# Autodesk Inventor assembly: solar_harvester_v2
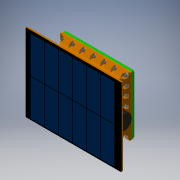
[picture p0: Inventor's stored thumbnail of the model, 180x180]
Saved by Autodesk Inventor 2018 (Build 220112000, 112)
## iProperties
Created: 2019-07-24
Part Number: solar_harvester_v2
Document SubType Name: Assembly
Designer: ZEUSLAP
Author: ZEUSLAP
## Documents named in this file (14)
- C:\data\solar-harvester\solar_harvester_136x110_CN3065_CGS.iam
- C:\data\solar-harvester\parts\sp16_waterproof_connector\sp16-2P_female_back_nut_type.iam
- C:\data\solar-harvester\parts\sp16_waterproof_connector\parts\nut.ipt
- C:\data\solar-harvester\parts\sp16_waterproof_connector\parts\rubber_washer.ipt
- C:\data\solar-harvester\enclosure\back\back_lid_CN3065_CGS.ipt
- C:\data\solar-harvester\parts\battery_holders\18650_battery_holder_CGS.ipt
- C:\data\solar-harvester\parts\18650_battery.ipt
- C:\data\solar-harvester\enclosure\back\charger_holder_CN3065.ipt
- C:\data\solar-harvester\enclosure\front\solar_panel_frame.ipt
- C:\data\solar-harvester\parts\panels\solar_panel_136x110mm.ipt
- C:\data\solar-harvester\parts\chargers\CN3065_solar_charger_board_Shrinkwrap.ipt
- C:\Users\ZEUSLAP\Documents\Inventor\Content Center Files\R2018\en-US\SFS EN ISO 7045 Z\EN ISO 7045 - M3 x 8 - 4.8 - Z(3).ipt
- C:\Users\ZEUSLAP\Documents\Inventor\Content Center Files\R2018\en-US\ISO 4035(2)\ISO 4035 - M3 - ISO.ipt
- C:\Users\ZEUSLAP\Documents\Inventor\Content Center Files\R2018\en-US\ISO 7049 - C-Z(2)\ISO 7049 - ST 2.9 x 6.5 - C - Z.ipt
## Components (59 placed, 13 different names)
1. solar_panel_136x110mm:1 — Mate:43, Mate:44, Angle:2, Mate:45
2. solar_panel_frame_136x110:1 — Mate:36, Mate:37, Mate:38, Angle:1, Mate:43, Mate:44, Angle:2, Mate:45, Mate:50, Mate:51, Mate:52, Mate:53, Angle:5, Mate:54, Mate:55, Mate:103, Mate:105, Mate:107, Mate:109, Mate:111, Mate:113, Mate:115, Mate:117, Mate:119, Mate:121, Mate:123, Mate:125, Mate:127, Mate:129, Mate:131, Mate:133, Mate:135, Mate:137, Mate:139, Mate:141, Mate:143, Mate:145, Mate:147
3. SP16-2P, female, back nut type:1 [sub-assembly] — Mate:31, Mate:32, Mate:34, Mate:37
4. nut:1 — Mate:32, Mate:38, Angle:1
5. rubber_washer:1 — Mate:31, Mate:34, Mate:36
6. back_lid_CN3065_CGS:1 — Mate:20, Mate:21, Mate:35, Mate:39, Angle:3, Angle:4, Mate:46, Mate:47, Mate:48, Mate:49, Mate:50, Mate:51, Mate:52, Mate:53, Mate:56, Mate:57, Mate:58, Mate:59, Mate:60, Mate:61, Mate:62, Mate:63, Mate:64, Mate:65, Mate:66, Mate:67, Mate:68, Mate:69, Mate:70, Mate:71, Mate:72, Mate:73, Mate:74, Mate:75, Mate:76, Mate:77, Mate:78, Mate:79, Mate:80, Mate:81, Mate:82, Mate:83, Mate:84, Mate:85, Mate:86, Mate:87, Mate:88, Mate:89, Mate:90, Mate:91, Mate:92, Mate:93, Mate:94, Mate:95, Mate:96, Mate:97, Mate:98, Mate:99, Mate:100, Mate:101, Mate:152
7. 18650_battery_holder_CGS:1 — Mate:22, Mate:23, Mate:35, Angle:3, Mate:46, Mate:153
8. 18650_battery:1 — Mate:22, Mate:23
9. CN3065_solar_charger_board:1 — Mate:39, Angle:4, Mate:48, Mate:49
10. charger_holder_CN3065:1 — Mate:20, Mate:21, Mate:47, Mate:148, Mate:149, Mate:150, Mate:151
11. SFS EN ISO 7045 Z M3 x 8 - 4.8 - Z:1 — Mate:56, Mate:57, Mate:108
12. SFS EN ISO 7045 Z M3 x 8 - 4.8 - Z:2 — Mate:58, Mate:59, Mate:118
13. SFS EN ISO 7045 Z M3 x 8 - 4.8 - Z:3 — Mate:60, Mate:61, Mate:122
14. SFS EN ISO 7045 Z M3 x 8 - 4.8 - Z:4 — Mate:62, Mate:63, Mate:138
15. SFS EN ISO 7045 Z M3 x 8 - 4.8 - Z:5 — Mate:64, Mate:65, Mate:142
16. SFS EN ISO 7045 Z M3 x 8 - 4.8 - Z:6 — Mate:66, Mate:67, Mate:136
17. SFS EN ISO 7045 Z M3 x 8 - 4.8 - Z:7 — Mate:68, Mate:69, Mate:132
18. SFS EN ISO 7045 Z M3 x 8 - 4.8 - Z:8 — Mate:70, Mate:71, Mate:128
19. SFS EN ISO 7045 Z M3 x 8 - 4.8 - Z:9 — Mate:72, Mate:73, Mate:124
20. SFS EN ISO 7045 Z M3 x 8 - 4.8 - Z:10 — Mate:74, Mate:75, Mate:112
21. SFS EN ISO 7045 Z M3 x 8 - 4.8 - Z:11 — Mate:76, Mate:77, Mate:104
22. SFS EN ISO 7045 Z M3 x 8 - 4.8 - Z:12 — Mate:78, Mate:79, Mate:102
23. SFS EN ISO 7045 Z M3 x 8 - 4.8 - Z:13 — Mate:80, Mate:81, Mate:106
24. SFS EN ISO 7045 Z M3 x 8 - 4.8 - Z:14 — Mate:82, Mate:83, Mate:110
25. SFS EN ISO 7045 Z M3 x 8 - 4.8 - Z:15 — Mate:84, Mate:85, Mate:114
26. SFS EN ISO 7045 Z M3 x 8 - 4.8 - Z:16 — Mate:86, Mate:87, Mate:126
27. SFS EN ISO 7045 Z M3 x 8 - 4.8 - Z:17 — Mate:88, Mate:89, Mate:130
28. SFS EN ISO 7045 Z M3 x 8 - 4.8 - Z:18 — Mate:90, Mate:91, Mate:134
29. SFS EN ISO 7045 Z M3 x 8 - 4.8 - Z:19 — Mate:92, Mate:93, Mate:144
30. SFS EN ISO 7045 Z M3 x 8 - 4.8 - Z:20 — Mate:94, Mate:95, Mate:140
31. SFS EN ISO 7045 Z M3 x 8 - 4.8 - Z:21 — Mate:96, Mate:97, Mate:146
32. SFS EN ISO 7045 Z M3 x 8 - 4.8 - Z:22 — Mate:98, Mate:99, Mate:120
33. SFS EN ISO 7045 Z M3 x 8 - 4.8 - Z:23 — Mate:100, Mate:101, Mate:116
34. ISO 4035 M3:1 — Mate:102, Mate:103
35. ISO 4035 M3:2 — Mate:104, Mate:105
36. ISO 4035 M3:3 — Mate:106, Mate:107
37. ISO 4035 M3:4 — Mate:108, Mate:109
38. ISO 4035 M3:5 — Mate:110, Mate:111
39. ISO 4035 M3:6 — Mate:112, Mate:113
40. ISO 4035 M3:7 — Mate:114, Mate:115
41. ISO 4035 M3:8 — Mate:116, Mate:117
42. ISO 4035 M3:9 — Mate:118, Mate:119
43. ISO 4035 M3:10 — Mate:120, Mate:121
44. ISO 4035 M3:11 — Mate:122, Mate:123
45. ISO 4035 M3:12 — Mate:124, Mate:125
46. ISO 4035 M3:13 — Mate:126, Mate:127
47. ISO 4035 M3:14 — Mate:128, Mate:129
48. ISO 4035 M3:15 — Mate:130, Mate:131
49. ISO 4035 M3:16 — Mate:132, Mate:133
50. ISO 4035 M3:17 — Mate:134, Mate:135
51. ISO 4035 M3:18 — Mate:136, Mate:137
52. ISO 4035 M3:19 — Mate:138, Mate:139
53. ISO 4035 M3:20 — Mate:140, Mate:141
54. ISO 4035 M3:21 — Mate:142, Mate:143
55. ISO 4035 M3:22 — Mate:144, Mate:145
56. ISO 4035 M3:23 — Mate:146, Mate:147
57. ISO 7049 - C-Z ST 2.9 x 6.5 - C - Z:1 — Mate:148, Mate:149
58. ISO 7049 - C-Z ST 2.9 x 6.5 - C - Z:2 — Mate:150, Mate:151
59. ISO 7049 - C-Z ST 2.9 x 6.5 - C - Z:3 — Mate:152, Mate:153
## Relationships (128: Mate 123, Angle 5)
- Mate:20: back_lid_CN3065_CGS:1 ↔ charger_holder_CN3065:1
- Mate:21: back_lid_CN3065_CGS:1 ↔ charger_holder_CN3065:1
- Mate:22: 18650_battery_holder_CGS:1 ↔ 18650_battery:1
- Mate:23: 18650_battery_holder_CGS:1 ↔ 18650_battery:1
- Mate:31: SP16-2P, female, back nut type:1 ↔ rubber_washer:1
- Mate:32: SP16-2P, female, back nut type:1 ↔ nut:1
- Mate:34: SP16-2P, female, back nut type:1 ↔ rubber_washer:1
- Mate:35: back_lid_CN3065_CGS:1 ↔ 18650_battery_holder_CGS:1
- Mate:36: solar_panel_frame_136x110:1 ↔ rubber_washer:1
- Mate:37: solar_panel_frame_136x110:1 ↔ SP16-2P, female, back nut type:1
- Mate:38: solar_panel_frame_136x110:1 ↔ nut:1
- Angle:1 (0 deg): solar_panel_frame_136x110:1 ↔ nut:1
- Mate:39: back_lid_CN3065_CGS:1 ↔ CN3065_solar_charger_board:1
- Mate:43: solar_panel_136x110mm:1 ↔ solar_panel_frame_136x110:1
- Mate:44: solar_panel_136x110mm:1 ↔ solar_panel_frame_136x110:1
- Angle:2 (180 deg): solar_panel_136x110mm:1 ↔ solar_panel_frame_136x110:1
- Mate:45: solar_panel_136x110mm:1 ↔ solar_panel_frame_136x110:1
- Angle:3 (0 deg): back_lid_CN3065_CGS:1 ↔ 18650_battery_holder_CGS:1
- Angle:4 (180 deg): back_lid_CN3065_CGS:1 ↔ CN3065_solar_charger_board:1
- Mate:46: back_lid_CN3065_CGS:1 ↔ 18650_battery_holder_CGS:1
- Mate:47: back_lid_CN3065_CGS:1 ↔ charger_holder_CN3065:1
- Mate:48 (1 mm): back_lid_CN3065_CGS:1 ↔ CN3065_solar_charger_board:1
- Mate:49 (1 mm): back_lid_CN3065_CGS:1 ↔ CN3065_solar_charger_board:1
- Mate:50: solar_panel_frame_136x110:1 ↔ back_lid_CN3065_CGS:1
- Mate:51: solar_panel_frame_136x110:1 ↔ back_lid_CN3065_CGS:1
- Mate:52: solar_panel_frame_136x110:1 ↔ back_lid_CN3065_CGS:1
- Mate:53: solar_panel_frame_136x110:1 ↔ back_lid_CN3065_CGS:1
- Angle:5 (90 deg): solar_panel_frame_136x110:1
- Mate:54: solar_panel_frame_136x110:1
- Mate:55: solar_panel_frame_136x110:1
- Mate:56: back_lid_CN3065_CGS:1 ↔ SFS EN ISO 7045 Z M3 x 8 - 4.8 - Z:1
- Mate:57: back_lid_CN3065_CGS:1 ↔ SFS EN ISO 7045 Z M3 x 8 - 4.8 - Z:1
- Mate:58: back_lid_CN3065_CGS:1 ↔ SFS EN ISO 7045 Z M3 x 8 - 4.8 - Z:2
- Mate:59: back_lid_CN3065_CGS:1 ↔ SFS EN ISO 7045 Z M3 x 8 - 4.8 - Z:2
- Mate:60: back_lid_CN3065_CGS:1 ↔ SFS EN ISO 7045 Z M3 x 8 - 4.8 - Z:3
- Mate:61: back_lid_CN3065_CGS:1 ↔ SFS EN ISO 7045 Z M3 x 8 - 4.8 - Z:3
- Mate:62: back_lid_CN3065_CGS:1 ↔ SFS EN ISO 7045 Z M3 x 8 - 4.8 - Z:4
- Mate:63: back_lid_CN3065_CGS:1 ↔ SFS EN ISO 7045 Z M3 x 8 - 4.8 - Z:4
- Mate:64: back_lid_CN3065_CGS:1 ↔ SFS EN ISO 7045 Z M3 x 8 - 4.8 - Z:5
- Mate:65: back_lid_CN3065_CGS:1 ↔ SFS EN ISO 7045 Z M3 x 8 - 4.8 - Z:5
- Mate:66: back_lid_CN3065_CGS:1 ↔ SFS EN ISO 7045 Z M3 x 8 - 4.8 - Z:6
- Mate:67: back_lid_CN3065_CGS:1 ↔ SFS EN ISO 7045 Z M3 x 8 - 4.8 - Z:6
- Mate:68: back_lid_CN3065_CGS:1 ↔ SFS EN ISO 7045 Z M3 x 8 - 4.8 - Z:7
- Mate:69: back_lid_CN3065_CGS:1 ↔ SFS EN ISO 7045 Z M3 x 8 - 4.8 - Z:7
- Mate:70: back_lid_CN3065_CGS:1 ↔ SFS EN ISO 7045 Z M3 x 8 - 4.8 - Z:8
- Mate:71: back_lid_CN3065_CGS:1 ↔ SFS EN ISO 7045 Z M3 x 8 - 4.8 - Z:8
- Mate:72: back_lid_CN3065_CGS:1 ↔ SFS EN ISO 7045 Z M3 x 8 - 4.8 - Z:9
- Mate:73: back_lid_CN3065_CGS:1 ↔ SFS EN ISO 7045 Z M3 x 8 - 4.8 - Z:9
- Mate:74: back_lid_CN3065_CGS:1 ↔ SFS EN ISO 7045 Z M3 x 8 - 4.8 - Z:10
- Mate:75: back_lid_CN3065_CGS:1 ↔ SFS EN ISO 7045 Z M3 x 8 - 4.8 - Z:10
- Mate:76: back_lid_CN3065_CGS:1 ↔ SFS EN ISO 7045 Z M3 x 8 - 4.8 - Z:11
- Mate:77: back_lid_CN3065_CGS:1 ↔ SFS EN ISO 7045 Z M3 x 8 - 4.8 - Z:11
- Mate:78: back_lid_CN3065_CGS:1 ↔ SFS EN ISO 7045 Z M3 x 8 - 4.8 - Z:12
- Mate:79: back_lid_CN3065_CGS:1 ↔ SFS EN ISO 7045 Z M3 x 8 - 4.8 - Z:12
- Mate:80: back_lid_CN3065_CGS:1 ↔ SFS EN ISO 7045 Z M3 x 8 - 4.8 - Z:13
- Mate:81: back_lid_CN3065_CGS:1 ↔ SFS EN ISO 7045 Z M3 x 8 - 4.8 - Z:13
- Mate:82: back_lid_CN3065_CGS:1 ↔ SFS EN ISO 7045 Z M3 x 8 - 4.8 - Z:14
- Mate:83: back_lid_CN3065_CGS:1 ↔ SFS EN ISO 7045 Z M3 x 8 - 4.8 - Z:14
- Mate:84: back_lid_CN3065_CGS:1 ↔ SFS EN ISO 7045 Z M3 x 8 - 4.8 - Z:15
- Mate:85: back_lid_CN3065_CGS:1 ↔ SFS EN ISO 7045 Z M3 x 8 - 4.8 - Z:15
- Mate:86: back_lid_CN3065_CGS:1 ↔ SFS EN ISO 7045 Z M3 x 8 - 4.8 - Z:16
- Mate:87: back_lid_CN3065_CGS:1 ↔ SFS EN ISO 7045 Z M3 x 8 - 4.8 - Z:16
- Mate:88: back_lid_CN3065_CGS:1 ↔ SFS EN ISO 7045 Z M3 x 8 - 4.8 - Z:17
- Mate:89: back_lid_CN3065_CGS:1 ↔ SFS EN ISO 7045 Z M3 x 8 - 4.8 - Z:17
- Mate:90: back_lid_CN3065_CGS:1 ↔ SFS EN ISO 7045 Z M3 x 8 - 4.8 - Z:18
- Mate:91: back_lid_CN3065_CGS:1 ↔ SFS EN ISO 7045 Z M3 x 8 - 4.8 - Z:18
- Mate:92: back_lid_CN3065_CGS:1 ↔ SFS EN ISO 7045 Z M3 x 8 - 4.8 - Z:19
- Mate:93: back_lid_CN3065_CGS:1 ↔ SFS EN ISO 7045 Z M3 x 8 - 4.8 - Z:19
- Mate:94: back_lid_CN3065_CGS:1 ↔ SFS EN ISO 7045 Z M3 x 8 - 4.8 - Z:20
- Mate:95: back_lid_CN3065_CGS:1 ↔ SFS EN ISO 7045 Z M3 x 8 - 4.8 - Z:20
- Mate:96: back_lid_CN3065_CGS:1 ↔ SFS EN ISO 7045 Z M3 x 8 - 4.8 - Z:21
- Mate:97: back_lid_CN3065_CGS:1 ↔ SFS EN ISO 7045 Z M3 x 8 - 4.8 - Z:21
- Mate:98: back_lid_CN3065_CGS:1 ↔ SFS EN ISO 7045 Z M3 x 8 - 4.8 - Z:22
- Mate:99: back_lid_CN3065_CGS:1 ↔ SFS EN ISO 7045 Z M3 x 8 - 4.8 - Z:22
- Mate:100: back_lid_CN3065_CGS:1 ↔ SFS EN ISO 7045 Z M3 x 8 - 4.8 - Z:23
- Mate:101: back_lid_CN3065_CGS:1 ↔ SFS EN ISO 7045 Z M3 x 8 - 4.8 - Z:23
- Mate:102: SFS EN ISO 7045 Z M3 x 8 - 4.8 - Z:12 ↔ ISO 4035 M3:1
- Mate:103: solar_panel_frame_136x110:1 ↔ ISO 4035 M3:1
- Mate:104: SFS EN ISO 7045 Z M3 x 8 - 4.8 - Z:11 ↔ ISO 4035 M3:2
- Mate:105: solar_panel_frame_136x110:1 ↔ ISO 4035 M3:2
- Mate:106: SFS EN ISO 7045 Z M3 x 8 - 4.8 - Z:13 ↔ ISO 4035 M3:3
- Mate:107: solar_panel_frame_136x110:1 ↔ ISO 4035 M3:3
- Mate:108: SFS EN ISO 7045 Z M3 x 8 - 4.8 - Z:1 ↔ ISO 4035 M3:4
- Mate:109: solar_panel_frame_136x110:1 ↔ ISO 4035 M3:4
- Mate:110: SFS EN ISO 7045 Z M3 x 8 - 4.8 - Z:14 ↔ ISO 4035 M3:5
- Mate:111: solar_panel_frame_136x110:1 ↔ ISO 4035 M3:5
- Mate:112: SFS EN ISO 7045 Z M3 x 8 - 4.8 - Z:10 ↔ ISO 4035 M3:6
- Mate:113: solar_panel_frame_136x110:1 ↔ ISO 4035 M3:6
- Mate:114: SFS EN ISO 7045 Z M3 x 8 - 4.8 - Z:15 ↔ ISO 4035 M3:7
- Mate:115: solar_panel_frame_136x110:1 ↔ ISO 4035 M3:7
- Mate:116: SFS EN ISO 7045 Z M3 x 8 - 4.8 - Z:23 ↔ ISO 4035 M3:8
- Mate:117: solar_panel_frame_136x110:1 ↔ ISO 4035 M3:8
- Mate:118: SFS EN ISO 7045 Z M3 x 8 - 4.8 - Z:2 ↔ ISO 4035 M3:9
- Mate:119: solar_panel_frame_136x110:1 ↔ ISO 4035 M3:9
- Mate:120: SFS EN ISO 7045 Z M3 x 8 - 4.8 - Z:22 ↔ ISO 4035 M3:10
- Mate:121: solar_panel_frame_136x110:1 ↔ ISO 4035 M3:10
- Mate:122: SFS EN ISO 7045 Z M3 x 8 - 4.8 - Z:3 ↔ ISO 4035 M3:11
- Mate:123: solar_panel_frame_136x110:1 ↔ ISO 4035 M3:11
- Mate:124: SFS EN ISO 7045 Z M3 x 8 - 4.8 - Z:9 ↔ ISO 4035 M3:12
- Mate:125: solar_panel_frame_136x110:1 ↔ ISO 4035 M3:12
- Mate:126: SFS EN ISO 7045 Z M3 x 8 - 4.8 - Z:16 ↔ ISO 4035 M3:13
- Mate:127: solar_panel_frame_136x110:1 ↔ ISO 4035 M3:13
- Mate:128: SFS EN ISO 7045 Z M3 x 8 - 4.8 - Z:8 ↔ ISO 4035 M3:14
- Mate:129: solar_panel_frame_136x110:1 ↔ ISO 4035 M3:14
- Mate:130: SFS EN ISO 7045 Z M3 x 8 - 4.8 - Z:17 ↔ ISO 4035 M3:15
- Mate:131: solar_panel_frame_136x110:1 ↔ ISO 4035 M3:15
- Mate:132: SFS EN ISO 7045 Z M3 x 8 - 4.8 - Z:7 ↔ ISO 4035 M3:16
- Mate:133: solar_panel_frame_136x110:1 ↔ ISO 4035 M3:16
- Mate:134: SFS EN ISO 7045 Z M3 x 8 - 4.8 - Z:18 ↔ ISO 4035 M3:17
- Mate:135: solar_panel_frame_136x110:1 ↔ ISO 4035 M3:17
- Mate:136: SFS EN ISO 7045 Z M3 x 8 - 4.8 - Z:6 ↔ ISO 4035 M3:18
- Mate:137: solar_panel_frame_136x110:1 ↔ ISO 4035 M3:18
- Mate:138: SFS EN ISO 7045 Z M3 x 8 - 4.8 - Z:4 ↔ ISO 4035 M3:19
- Mate:139: solar_panel_frame_136x110:1 ↔ ISO 4035 M3:19
- Mate:140: SFS EN ISO 7045 Z M3 x 8 - 4.8 - Z:20 ↔ ISO 4035 M3:20
- Mate:141: solar_panel_frame_136x110:1 ↔ ISO 4035 M3:20
- Mate:142: SFS EN ISO 7045 Z M3 x 8 - 4.8 - Z:5 ↔ ISO 4035 M3:21
- Mate:143: solar_panel_frame_136x110:1 ↔ ISO 4035 M3:21
- Mate:144: SFS EN ISO 7045 Z M3 x 8 - 4.8 - Z:19 ↔ ISO 4035 M3:22
- Mate:145: solar_panel_frame_136x110:1 ↔ ISO 4035 M3:22
- Mate:146: SFS EN ISO 7045 Z M3 x 8 - 4.8 - Z:21 ↔ ISO 4035 M3:23
- Mate:147: solar_panel_frame_136x110:1 ↔ ISO 4035 M3:23
- Mate:148: charger_holder_CN3065:1 ↔ ISO 7049 - C-Z ST 2.9 x 6.5 - C - Z:1
- Mate:149: charger_holder_CN3065:1 ↔ ISO 7049 - C-Z ST 2.9 x 6.5 - C - Z:1
- Mate:150: charger_holder_CN3065:1 ↔ ISO 7049 - C-Z ST 2.9 x 6.5 - C - Z:2
- Mate:151: charger_holder_CN3065:1 ↔ ISO 7049 - C-Z ST 2.9 x 6.5 - C - Z:2
- Mate:152: back_lid_CN3065_CGS:1 ↔ ISO 7049 - C-Z ST 2.9 x 6.5 - C - Z:3
- Mate:153: 18650_battery_holder_CGS:1 ↔ ISO 7049 - C-Z ST 2.9 x 6.5 - C - Z:3
